# Autodesk Inventor assembly: trackey
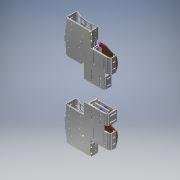
[picture p0: Inventor's stored thumbnail of the model, 180x180]
Saved by Autodesk Inventor 2018 (Build 220112000, 112)
## iProperties
Created: 2018-04-03
Part Number: trackey
Material: 一般
Document SubType Name: Assembly
Designer: NaMACHAN
Mass: 87.7582 g
Surface Area: 305.42 cm^2
Volume: 44.0784 cm^3
Density: 1.99096 g/cm^3
Author: NaMACHAN
## Documents named in this file (22)
- C:\Users\NaMACHAN\Dropbox\Project\original\Trackey\inventor\trackey.iam
- C:\Users\NaMACHAN\Dropbox\Project\original\Trackey\inventor\ball.ipt
- C:\Users\NaMACHAN\Dropbox\Project\original\Trackey\inventor\ball_cover.ipt
- C:\Users\NaMACHAN\Dropbox\Project\original\Trackey\inventor\trackball_base.ipt
- C:\Users\NaMACHAN\Dropbox\Project\original\Trackey\inventor\bearing_shaft.ipt
- C:\Users\NaMACHAN\Dropbox\Project\original\Trackey\inventor\bearing.ipt
- C:\Users\NaMACHAN\Dropbox\Project\original\Trackey\inventor\shaft_cover.ipt
- C:\Users\NaMACHAN\Dropbox\Project\original\Trackey\inventor\trackball_spacer.ipt
- C:\Users\NaMACHAN\Dropbox\Project\original\Trackey\inventor\sensor_cover.ipt
- C:\Users\NaMACHAN\Dropbox\Project\original\Trackey\inventor\sensor_sensorcover_spacer.ipt
- C:\Users\NaMACHAN\Dropbox\Project\original\Trackey\inventor\sensor_pcb.ipt
- C:\Users\NaMACHAN\Dropbox\Project\original\Trackey\inventor\trackball_cup.ipt
- C:\Users\NaMACHAN\Dropbox\Project\original\Trackey\inventor\base_plate.ipt
- C:\Users\NaMACHAN\Dropbox\Project\original\Trackey\inventor\key_plate.ipt
- C:\Users\NaMACHAN\Dropbox\Project\original\Trackey\inventor\main_key_cup.ipt
- C:\Users\NaMACHAN\Dropbox\Project\original\Trackey\inventor\palmrest_L_large.ipt
- C:\Users\NaMACHAN\Dropbox\Project\original\Trackey\inventor\palmrest_L_small.ipt
- C:\Users\NaMACHAN\Documents\palmrest_cup.ipt
- C:\Users\NaMACHAN\Documents\thumbkey_plate.ipt
- C:\Users\NaMACHAN\Dropbox\Project\original\Trackey\inventor\thumbkey_cup.ipt
- C:\Users\NaMACHAN\Documents\palmrest_rev2.ipt
- C:\Users\NaMACHAN\Documents\palmrest__left.ipt
## Components (56 placed, 21 different names)
1. ball:1 — メイト:17, メイト:18
2. ball_cover:1 — 挿入:6, メイト:19, 挿入:7, メイト:20, メイト:23, フラッシュ:1
3. trackball_base:1 — メイト:1, メイト:2, メイト:3, メイト:4, メイト:5, メイト:6, メイト:7, メイト:8, メイト:9, メイト:13, メイト:14, メイト:15, 挿入:1, メイト:16, メイト:17, メイト:22
4. bearing_shaft:1 — メイト:4, メイト:5, メイト:6, メイト:11
5. bearing_shaft:2 — メイト:7, メイト:8, メイト:9, メイト:10
6. bearing_shaft:3 — メイト:1, メイト:2, メイト:3, メイト:12
7. bearing:1 — メイト:10, メイト:14
8. bearing:2 — メイト:12, メイト:15
9. bearing:3 — メイト:11, メイト:13
10. shaft_cover:1 — 挿入:1, メイト:16, メイト:18, 挿入:2, 挿入:3, 挿入:4, 挿入:5
11. trackball_spacer:1 — 挿入:2
12. trackball_spacer:2 — 挿入:3
13. trackball_spacer:3 — 挿入:5, メイト:19
14. trackball_spacer:4 — 挿入:4, 挿入:6
15. sensor_cover:1 — 挿入:7, メイト:20, 挿入:8, 挿入:9
16. sensor_sensorcover_spacer:1 — 挿入:8, 挿入:10
17. sensor_sensorcover_spacer:2 — 挿入:9, メイト:21
18. sensor_pcb:1 — 挿入:10, メイト:21
19. trackball_cup:1 — メイト:22, メイト:23, フラッシュ:1, フラッシュ:2, フラッシュ:3, メイト:24, フラッシュ:4
20. base_plate:1 — フラッシュ:2, フラッシュ:3, メイト:24, フラッシュ:4, メイト:31, メイト:32, メイト:33, メイト:34, メイト:35, メイト:36, メイト:37, メイト:38, メイト:39, メイト:40, メイト:41, メイト:42, メイト:43, メイト:44, メイト:45, メイト:46, メイト:47, メイト:48, フラッシュ:22, メイト:53, フラッシュ:24, フラッシュ:25, フラッシュ:26, メイト:54, フラッシュ:49
21. key_plate:1 — メイト:25, フラッシュ:5, フラッシュ:6
22. main_key_cup:1 — メイト:25, フラッシュ:5, フラッシュ:6, メイト:31, メイト:32, メイト:33, フラッシュ:21
23. key_plate:2
24. main_key_cup:2 — メイト:34, メイト:39, メイト:40, フラッシュ:20, フラッシュ:21
25. key_plate:3
26. main_key_cup:3 — メイト:35, メイト:41, メイト:42, フラッシュ:19, フラッシュ:20
27. key_plate:4
28. main_key_cup:4 — メイト:36, メイト:43, メイト:44, フラッシュ:18, フラッシュ:19
29. key_plate:5
30. main_key_cup:5 — メイト:37, メイト:45, メイト:46, フラッシュ:17, フラッシュ:18
31. key_plate:6
32. main_key_cup:6 — メイト:38, メイト:47, メイト:48, フラッシュ:17, フラッシュ:22
33. palmrest_L_large:1 — フラッシュ:23, メイト:94, メイト:96
34. palmrest_L_small:1 — メイト:51, 挿入:12, メイト:95
35. palmrest_cup:1 — メイト:51, フラッシュ:23, メイト:53, フラッシュ:24, フラッシュ:25, メイト:97
36. base_plate:2 — フラッシュ:26, メイト:54, フラッシュ:29, フラッシュ:30, メイト:59, メイト:66, メイト:67, メイト:68, メイト:69, メイト:70, メイト:71, メイト:72, メイト:74, メイト:75, メイト:76, メイト:77, メイト:78, メイト:79, メイト:80, メイト:81, メイト:82, メイト:83, メイト:84, メイト:85, フラッシュ:48, フラッシュ:49, フラッシュ:50, フラッシュ:51, メイト:86
37. palmrest_L_large:2 — 挿入:13, メイト:99
38. palmrest_L_small:2 — メイト:98, メイト:100
39. palmrest_cup:2 — フラッシュ:29, フラッシュ:30, メイト:59, メイト:101
40. key_plate:7
41. main_key_cup:7 — メイト:66, メイト:74, メイト:81, フラッシュ:43, フラッシュ:48
42. key_plate:8
43. main_key_cup:8 — メイト:67, メイト:68, メイト:77, メイト:78, フラッシュ:45, フラッシュ:46
44. key_plate:9
45. main_key_cup:9 — メイト:69, メイト:79, メイト:80, フラッシュ:46, フラッシュ:47
46. key_plate:10
47. main_key_cup:10 — メイト:70, メイト:75, メイト:76, フラッシュ:44, フラッシュ:45
48. key_plate:11
49. main_key_cup:11 — メイト:71, メイト:82, メイト:83, フラッシュ:43, フラッシュ:44
50. key_plate:12
51. main_key_cup:12 — メイト:72, メイト:84, メイト:85, フラッシュ:47
52. thumbkey_plate:1 — メイト:88, フラッシュ:52, フラッシュ:55
53. thumbkey_plate:2 — メイト:87, フラッシュ:53, フラッシュ:54
54. thumbkey_cup:1 — フラッシュ:50, フラッシュ:51, メイト:86, メイト:87, メイト:88, フラッシュ:52, フラッシュ:53, フラッシュ:54, フラッシュ:55
55. palmrest_rev2:2 — 挿入:12, メイト:94, メイト:95, メイト:96, メイト:97
56. palmrest__left:1 — 挿入:13, メイト:98, メイト:99, メイト:100, メイト:101
## Relationships (155: Mate 89, Flush 54, Insert 12)
- メイト:1 [Mate] (1 mm): trackball_base:1 ↔ bearing_shaft:3
- メイト:2 [Mate] (1 mm): trackball_base:1 ↔ bearing_shaft:3
- メイト:3 [Mate]: trackball_base:1 ↔ bearing_shaft:3
- メイト:4 [Mate] (1 mm): trackball_base:1 ↔ bearing_shaft:1
- メイト:5 [Mate] (1 mm): trackball_base:1 ↔ bearing_shaft:1
- メイト:6 [Mate]: trackball_base:1 ↔ bearing_shaft:1
- メイト:7 [Mate] (1 mm): trackball_base:1 ↔ bearing_shaft:2
- メイト:8 [Mate] (1 mm): trackball_base:1 ↔ bearing_shaft:2
- メイト:9 [Mate]: trackball_base:1 ↔ bearing_shaft:2
- メイト:10 [Mate]: bearing_shaft:2 ↔ bearing:1
- メイト:11 [Mate]: bearing_shaft:1 ↔ bearing:3
- メイト:12 [Mate]: bearing_shaft:3 ↔ bearing:2
- メイト:13 [Mate] (0.75 mm): trackball_base:1 ↔ bearing:3
- メイト:14 [Mate] (0.75 mm): trackball_base:1 ↔ bearing:1
- メイト:15 [Mate] (0.75 mm): trackball_base:1 ↔ bearing:2
- 挿入:1 [Insert]: trackball_base:1 ↔ shaft_cover:1
- メイト:16 [Mate]: trackball_base:1 ↔ shaft_cover:1
- メイト:17 [Mate]: ball:1 ↔ trackball_base:1
- メイト:18 [Mate] (6.3 mm): ball:1 ↔ shaft_cover:1
- 挿入:2 [Insert]: shaft_cover:1 ↔ trackball_spacer:1
- 挿入:3 [Insert]: shaft_cover:1 ↔ trackball_spacer:2
- 挿入:4 [Insert]: shaft_cover:1 ↔ trackball_spacer:4
- 挿入:5 [Insert]: shaft_cover:1 ↔ trackball_spacer:3
- 挿入:6 [Insert]: ball_cover:1 ↔ trackball_spacer:4
- メイト:19 [Mate]: ball_cover:1 ↔ trackball_spacer:3
- 挿入:7 [Insert]: ball_cover:1 ↔ sensor_cover:1
- メイト:20 [Mate]: ball_cover:1 ↔ sensor_cover:1
- 挿入:8 [Insert]: sensor_cover:1 ↔ sensor_sensorcover_spacer:1
- 挿入:9 [Insert]: sensor_cover:1 ↔ sensor_sensorcover_spacer:2
- 挿入:10 [Insert]: sensor_sensorcover_spacer:1 ↔ sensor_pcb:1
- メイト:21 [Mate]: sensor_sensorcover_spacer:2 ↔ sensor_pcb:1
- メイト:22 [Mate] (10 mm): trackball_base:1 ↔ trackball_cup:1
- メイト:23 [Mate]: ball_cover:1 ↔ trackball_cup:1
- フラッシュ:1 [Flush]: ball_cover:1 ↔ trackball_cup:1
- フラッシュ:2 [Flush]: trackball_cup:1 ↔ base_plate:1
- フラッシュ:3 [Flush]: trackball_cup:1 ↔ base_plate:1
- メイト:24 [Mate]: trackball_cup:1 ↔ base_plate:1
- フラッシュ:4 [Flush] (-10 mm): trackball_cup:1 ↔ base_plate:1
- メイト:25 [Mate]: key_plate:1 ↔ main_key_cup:1
- フラッシュ:5 [Flush]: key_plate:1 ↔ main_key_cup:1
- フラッシュ:6 [Flush] (-15 mm): key_plate:1 ↔ main_key_cup:1
- [Mate]: key_plate:2 ↔ main_key_cup:2
- [Flush]: key_plate:2 ↔ main_key_cup:2
- [Flush] (-15 mm): key_plate:2 ↔ main_key_cup:2
- [Mate]: key_plate:3 ↔ main_key_cup:3
- [Flush]: key_plate:3 ↔ main_key_cup:3
- [Flush] (-15 mm): key_plate:3 ↔ main_key_cup:3
- [Mate]: key_plate:4 ↔ main_key_cup:4
- [Flush]: key_plate:4 ↔ main_key_cup:4
- [Flush] (-15 mm): key_plate:4 ↔ main_key_cup:4
- [Mate]: key_plate:5 ↔ main_key_cup:5
- [Flush]: key_plate:5 ↔ main_key_cup:5
- [Flush] (-15 mm): key_plate:5 ↔ main_key_cup:5
- [Mate]: key_plate:6 ↔ main_key_cup:6
- [Flush]: key_plate:6 ↔ main_key_cup:6
- [Flush] (-15 mm): key_plate:6 ↔ main_key_cup:6
- メイト:31 [Mate] (1 mm): base_plate:1 ↔ main_key_cup:1
- メイト:32 [Mate] (1 mm): base_plate:1 ↔ main_key_cup:1
- メイト:33 [Mate]: base_plate:1 ↔ main_key_cup:1
- メイト:34 [Mate]: base_plate:1 ↔ main_key_cup:2
- メイト:35 [Mate]: base_plate:1 ↔ main_key_cup:3
- メイト:36 [Mate]: base_plate:1 ↔ main_key_cup:4
- メイト:37 [Mate]: base_plate:1 ↔ main_key_cup:5
- メイト:38 [Mate]: base_plate:1 ↔ main_key_cup:6
- メイト:39 [Mate] (1 mm): base_plate:1 ↔ main_key_cup:2
- メイト:40 [Mate] (1 mm): base_plate:1 ↔ main_key_cup:2
- メイト:41 [Mate] (1 mm): base_plate:1 ↔ main_key_cup:3
- メイト:42 [Mate] (1 mm): base_plate:1 ↔ main_key_cup:3
- メイト:43 [Mate] (1 mm): base_plate:1 ↔ main_key_cup:4
- メイト:44 [Mate] (1 mm): base_plate:1 ↔ main_key_cup:4
- メイト:45 [Mate] (1 mm): base_plate:1 ↔ main_key_cup:5
- メイト:46 [Mate] (1 mm): base_plate:1 ↔ main_key_cup:5
- メイト:47 [Mate] (1 mm): base_plate:1 ↔ main_key_cup:6
- メイト:48 [Mate] (1 mm): base_plate:1 ↔ main_key_cup:6
- フラッシュ:17 [Flush]: main_key_cup:5 ↔ main_key_cup:6
- フラッシュ:18 [Flush] (5 mm): main_key_cup:4 ↔ main_key_cup:5
- フラッシュ:19 [Flush] (2 mm): main_key_cup:3 ↔ main_key_cup:4
- フラッシュ:20 [Flush] (3 mm): main_key_cup:2 ↔ main_key_cup:3
- フラッシュ:21 [Flush] (2 mm): main_key_cup:1 ↔ main_key_cup:2
- フラッシュ:22 [Flush] (-3 mm): base_plate:1 ↔ main_key_cup:6
- メイト:51 [Mate]: palmrest_L_small:1 ↔ palmrest_cup:1
- フラッシュ:23 [Flush] (-5 mm): palmrest_L_large:1 ↔ palmrest_cup:1
- メイト:53 [Mate]: base_plate:1 ↔ palmrest_cup:1
- フラッシュ:24 [Flush] (-10 mm): base_plate:1 ↔ palmrest_cup:1
- フラッシュ:25 [Flush]: base_plate:1 ↔ palmrest_cup:1
- フラッシュ:26 [Flush]: base_plate:1 ↔ base_plate:2
- メイト:54 [Mate] (150 mm): base_plate:1 ↔ base_plate:2
- [Mate]: palmrest_L_small:2 ↔ palmrest_cup:2
- [Flush] (-5 mm): palmrest_L_large:2 ↔ palmrest_cup:2
- フラッシュ:29 [Flush] (-10 mm): base_plate:2 ↔ palmrest_cup:2
- フラッシュ:30 [Flush]: base_plate:2 ↔ palmrest_cup:2
- メイト:59 [Mate]: base_plate:2 ↔ palmrest_cup:2
- [Mate]: key_plate:7 ↔ main_key_cup:7
- [Flush]: key_plate:7 ↔ main_key_cup:7
- [Flush] (-15 mm): key_plate:7 ↔ main_key_cup:7
- [Mate]: key_plate:8 ↔ main_key_cup:8
- [Flush]: key_plate:8 ↔ main_key_cup:8
- [Flush] (-15 mm): key_plate:8 ↔ main_key_cup:8
- [Mate]: key_plate:9 ↔ main_key_cup:9
- [Flush]: key_plate:9 ↔ main_key_cup:9
- [Flush] (-15 mm): key_plate:9 ↔ main_key_cup:9
- [Mate]: key_plate:10 ↔ main_key_cup:10
- [Flush]: key_plate:10 ↔ main_key_cup:10
- [Flush] (-15 mm): key_plate:10 ↔ main_key_cup:10
- [Mate]: key_plate:11 ↔ main_key_cup:11
- [Flush]: key_plate:11 ↔ main_key_cup:11
- [Flush] (-15 mm): key_plate:11 ↔ main_key_cup:11
- [Mate]: key_plate:12 ↔ main_key_cup:12
- [Flush]: key_plate:12 ↔ main_key_cup:12
- [Flush] (-15 mm): key_plate:12 ↔ main_key_cup:12
- メイト:66 [Mate]: base_plate:2 ↔ main_key_cup:7
- メイト:67 [Mate]: base_plate:2 ↔ main_key_cup:8
- メイト:68 [Mate]: base_plate:2 ↔ main_key_cup:8
- メイト:69 [Mate]: base_plate:2 ↔ main_key_cup:9
- メイト:70 [Mate]: base_plate:2 ↔ main_key_cup:10
- メイト:71 [Mate]: base_plate:2 ↔ main_key_cup:11
- メイト:72 [Mate]: base_plate:2 ↔ main_key_cup:12
- メイト:74 [Mate] (1 mm): base_plate:2 ↔ main_key_cup:7
- メイト:75 [Mate] (1 mm): base_plate:2 ↔ main_key_cup:10
- メイト:76 [Mate] (1 mm): base_plate:2 ↔ main_key_cup:10
- メイト:77 [Mate] (1 mm): base_plate:2 ↔ main_key_cup:8
- メイト:78 [Mate] (1 mm): base_plate:2 ↔ main_key_cup:8
- メイト:79 [Mate] (1 mm): base_plate:2 ↔ main_key_cup:9
- メイト:80 [Mate] (1 mm): base_plate:2 ↔ main_key_cup:9
- メイト:81 [Mate] (1 mm): base_plate:2 ↔ main_key_cup:7
- メイト:82 [Mate] (1 mm): base_plate:2 ↔ main_key_cup:11
- メイト:83 [Mate] (1 mm): base_plate:2 ↔ main_key_cup:11
- メイト:84 [Mate] (1 mm): base_plate:2 ↔ main_key_cup:12
- メイト:85 [Mate] (1 mm): base_plate:2 ↔ main_key_cup:12
- フラッシュ:43 [Flush]: main_key_cup:7 ↔ main_key_cup:11
- フラッシュ:44 [Flush] (5 mm): main_key_cup:10 ↔ main_key_cup:11
- フラッシュ:45 [Flush] (2 mm): main_key_cup:8 ↔ main_key_cup:10
- フラッシュ:46 [Flush] (3 mm): main_key_cup:8 ↔ main_key_cup:9
- フラッシュ:47 [Flush] (2 mm): main_key_cup:9 ↔ main_key_cup:12
- フラッシュ:48 [Flush] (-3 mm): base_plate:2 ↔ main_key_cup:7
- フラッシュ:49 [Flush]: base_plate:1 ↔ base_plate:2
- フラッシュ:50 [Flush]: base_plate:2 ↔ thumbkey_cup:1
- フラッシュ:51 [Flush]: base_plate:2 ↔ thumbkey_cup:1
- メイト:86 [Mate]: base_plate:2 ↔ thumbkey_cup:1
- メイト:87 [Mate]: thumbkey_plate:2 ↔ thumbkey_cup:1
- メイト:88 [Mate]: thumbkey_plate:1 ↔ thumbkey_cup:1
- フラッシュ:52 [Flush] (3 mm): thumbkey_plate:1 ↔ thumbkey_cup:1
- フラッシュ:53 [Flush] (-3 mm): thumbkey_plate:2 ↔ thumbkey_cup:1
- フラッシュ:54 [Flush]: thumbkey_plate:2 ↔ thumbkey_cup:1
- フラッシュ:55 [Flush]: thumbkey_plate:1 ↔ thumbkey_cup:1
- 挿入:12 [Insert]: palmrest_L_small:1 ↔ palmrest_rev2:2
- メイト:94 [Mate]: palmrest_L_large:1 ↔ palmrest_rev2:2
- メイト:95 [Mate]: palmrest_L_small:1 ↔ palmrest_rev2:2
- メイト:96 [Mate]: palmrest_L_large:1 ↔ palmrest_rev2:2
- メイト:97 [Mate] (20 mm): palmrest_cup:1 ↔ palmrest_rev2:2
- 挿入:13 [Insert]: palmrest_L_large:2 ↔ palmrest__left:1
- メイト:98 [Mate]: palmrest_L_small:2 ↔ palmrest__left:1
- メイト:99 [Mate]: palmrest_L_large:2 ↔ palmrest__left:1
- メイト:100 [Mate]: palmrest_L_small:2 ↔ palmrest__left:1
- メイト:101 [Mate] (20 mm): palmrest_cup:2 ↔ palmrest__left:1
## Named parameters: d347_d344 = 0 mm, d348_d345 = 0 mm, d349_d346 = -15 mm, d350_d344 = 0 mm, d351_d345 = 0 mm, d352_d346 = -15 mm, d353_d344 = 0 mm, d354_d345 = 0 mm, d355_d346 = -15 mm, d356_d344 = 0 mm, d357_d345 = 0 mm, d358_d346 = -15 mm, d359_d344 = 0 mm, d360_d345 = 0 mm, d361_d346 = -15 mm, d403_d390 = 0 mm, d404_d391 = -5 mm, d413_d344 = 0 mm, d414_d345 = 0 mm, d415_d346 = -15 mm, d416_d344 = 0 mm, d417_d345 = 0 mm, d418_d346 = -15 mm, d419_d344 = 0 mm, d420_d345 = 0 mm, d421_d346 = -15 mm, d422_d344 = 0 mm, d423_d345 = 0 mm, d424_d346 = -15 mm, d425_d344 = 0 mm, d426_d345 = 0 mm, d427_d346 = -15 mm, d428_d344 = 0 mm, d429_d345 = 0 mm, d430_d346 = -15 mm
